# Autodesk Inventor assembly: 276-2174
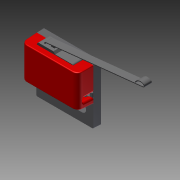
[picture p0: Inventor's stored thumbnail of the model, 180x180]
Saved by Autodesk Inventor 2013 (Build 170138000, 138)
## iProperties
Category: Sensors
Company: Autodesk Inc.
Created: 2012-04-10
Part Number: 276-2174
Document SubType Name: Assembly
Catalog Web Link: http://www.vexrobotics.com/products/accessories/sensors/276-2174.html
Vendor: VEX
Designer: Autodesk Inc.
Author: Autodesk Inc.
## Documents named in this file (4)
- C:\Data Folder\VEX 2012\VEX KOP Uploads\2013\Imperial\Sensors\Limit Switch.iam
- C:\Data Folder\VEX 2012\VEX KOP Uploads\2013\Imperial\Sensors\Components\LIMIT-SWITCH-MICROSWITCH.ipt
- C:\Data Folder\VEX 2012\VEX KOP Uploads\2013\Imperial\Sensors\Components\LIMIT-SWITCH-BOTTOM.ipt
- C:\Data Folder\VEX 2012\VEX KOP Uploads\2013\Imperial\Sensors\Components\LIMIT-SWITCH-TOP.ipt
## Components (3 placed, 3 different names)
1. LIMIT-SWITCH-MICROSWITCH:1 — Mate:5, Mate:6, Mate:7
2. LIMIT-SWITCH-BOTTOM:1 — Mate:1, Mate:2, Insert:1, Insert:2, Mate:5, Mate:6, Mate:7
3. LIMIT-SWITCH-TOP:1 — Insert:1, Insert:2
## Relationships (9: Mate 7, Insert 2)
- Mate:1: LIMIT-SWITCH-BOTTOM:1
- Mate:2: LIMIT-SWITCH-BOTTOM:1
- Mate:3
- Mate:4
- Insert:1: LIMIT-SWITCH-BOTTOM:1 ↔ LIMIT-SWITCH-TOP:1
- Insert:2: LIMIT-SWITCH-BOTTOM:1 ↔ LIMIT-SWITCH-TOP:1
- Mate:5: LIMIT-SWITCH-MICROSWITCH:1 ↔ LIMIT-SWITCH-BOTTOM:1
- Mate:6: LIMIT-SWITCH-MICROSWITCH:1 ↔ LIMIT-SWITCH-BOTTOM:1
- Mate:7: LIMIT-SWITCH-MICROSWITCH:1 ↔ LIMIT-SWITCH-BOTTOM:1
